# Autodesk Inventor assembly: Сборка1
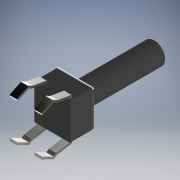
[picture p0: Inventor's stored thumbnail of the model, 180x180]
Saved by Autodesk Inventor 2021 (Build 250183000, 183)
## iProperties
Created: 2020-06-13
Part Number: Сборка1
Document SubType Name: Assembly
Designer: WEX
Author: WEX
## Documents named in this file (3)
- C:\Users\WEX\Desktop\PushButton_Files\Сборка1.iam
- C:\Users\WEX\Desktop\PushButton_Files\PushButton_Top.ipt
- C:\Users\WEX\Desktop\PushButton_Files\PushButton_Pins.ipt
## Components (5 placed, 2 different names)
1. PushButton_Top:1 — Жесткий:1, Жесткий:2, Жесткий:3, Жесткий:4
2. PushButton_Pins:1 — Жесткий:4
3. PushButton_Pins:2 — Жесткий:3
4. PushButton_Pins:3 — Жесткий:1
5. PushButton_Pins:4 — Жесткий:2
## Relationships (4: WeldJoint 4)
- Жесткий:1 [WeldJoint] (0.25 mm): PushButton_Top:1 ↔ PushButton_Pins:3
- Жесткий:2 [WeldJoint] (0.25 mm): PushButton_Top:1 ↔ PushButton_Pins:4
- Жесткий:3 [WeldJoint] (0.25 mm): PushButton_Top:1 ↔ PushButton_Pins:2
- Жесткий:4 [WeldJoint] (0.25 mm): PushButton_Top:1 ↔ PushButton_Pins:1
